# Autodesk Inventor assembly: axis5_6
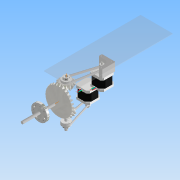
[picture p0: Inventor's stored thumbnail of the model, 180x180]
Saved by Autodesk Inventor 2020 (Build 240168000, 168)
## iProperties
Created: 2020-05-15
Part Number: axis5_6
Document SubType Name: Assembly
Designer: stefa
Author: stefa
## Documents named in this file (12)
- D:\github_gedeeld\BeerMinder\3D-model\axis5_6\axis5_6.iam
- D:\github_gedeeld\BeerMinder\3D-model\pulleys\tandriem32Tnaar16T_lengte240.ipt
- D:\github_gedeeld\BeerMinder\3D-model\pulleys\GT2 Timing Pulley 36T - 8mm as.ipt
- D:\github_gedeeld\BeerMinder\3D-model\stepper motors\42BYG Stepper Motor.ipt
- D:\github_gedeeld\BeerMinder\3D-model\pulleys\GT2 Pulley 16T - 5mm as.ipt
- D:\github_gedeeld\BeerMinder\3D-model\axis5_6\as_d8_l100.ipt
- D:\github_gedeeld\BeerMinder\3D-model\axis5_6\axis5_6\Design Accelerator\Bevel Gears1.iam
- D:\github_gedeeld\BeerMinder\3D-model\axis5_6\endeffector mount part.ipt
- D:\github_gedeeld\BeerMinder\3D-model\axis5_6\bovenarm - links.ipt
- D:\github_gedeeld\BeerMinder\3D-model\axis5_6\as naar endeffector.ipt
- D:\github_gedeeld\BeerMinder\3D-model\axis5_6\stepper spacer.ipt
- D:\github_gedeeld\BeerMinder\3D-model\axis5_6\axis5_6\Design Accelerator\Bevel Gear11.ipt
## Components (15 placed, 11 different names)
1. tandriem32Tnaar16T_lengte240:1 — Mate:5, Mate:6, Mate:21, Mate:22
2. GT2 Pulley 16T - 5mm as:1 — Mate:5, Mate:6, Mate:15, Mate:16
3. as_d8_l100:1 — Mate:20, Mate:23, Mate:26
4. tandriem32Tnaar16T_lengte240:2 — Mate:24, Mate:25
5. GT2 Pulley 16T - 5mm as:2 — Mate:17, Mate:18
6. Bevel Gears:1 [sub-assembly] — Mate:26, Mate:28, Mate:38, Mate:39
7. 42BYG Stepper Motor:2 — Mate:15, Mate:16, Flush:1, Mate:19, Mate:32, Angle:2, Mate:33, Mate:35, Mate:36, Mate:37
8. 42BYG Stepper Motor:3 — Mate:17, Mate:18, Flush:1, Mate:19, Angle:1
9. GT2 Timing Pulley 36T - 8mm as:3 — Mate:23, Mate:24, Mate:25
10. GT2 Timing Pulley 36T - 8mm as:4 — Mate:20, Mate:21, Mate:22
11. endeffector mount part:1 — Mate:27
12. bovenarm - links:1 — Mate:32, Angle:2, Mate:33, Angle:3, Mate:34
13. as naar endeffector:1 — Mate:27, Mate:28, Mate:29, Mate:30, Mate:31, Angle:1
14. stepper spacer:1 — Mate:34, Mate:35, Mate:36, Mate:37
15. Bevel Gear1:1 — Mate:38, Mate:39
## Relationships (33: Mate 29, Angle 3, Flush 1)
- Mate:5: tandriem32Tnaar16T_lengte240:1 ↔ GT2 Pulley 16T - 5mm as:1
- Mate:6 (0.5 mm): tandriem32Tnaar16T_lengte240:1 ↔ GT2 Pulley 16T - 5mm as:1
- [Mate]: tandriem32Tnaar16T_lengte240:2 ↔ GT2 Pulley 16T - 5mm as:2
- [Mate] (0.5 mm): tandriem32Tnaar16T_lengte240:2 ↔ GT2 Pulley 16T - 5mm as:2
- Mate:15: GT2 Pulley 16T - 5mm as:1 ↔ 42BYG Stepper Motor:2
- Mate:16 (2 mm): GT2 Pulley 16T - 5mm as:1 ↔ 42BYG Stepper Motor:2
- Mate:17 (2 mm): GT2 Pulley 16T - 5mm as:2 ↔ 42BYG Stepper Motor:3
- Mate:18: GT2 Pulley 16T - 5mm as:2 ↔ 42BYG Stepper Motor:3
- Flush:1: 42BYG Stepper Motor:2 ↔ 42BYG Stepper Motor:3
- Mate:19 (2 mm): 42BYG Stepper Motor:2 ↔ 42BYG Stepper Motor:3
- Mate:20: as_d8_l100:1 ↔ GT2 Timing Pulley 36T - 8mm as:4
- Mate:21: tandriem32Tnaar16T_lengte240:1 ↔ GT2 Timing Pulley 36T - 8mm as:4
- Mate:22 (0.5 mm): tandriem32Tnaar16T_lengte240:1 ↔ GT2 Timing Pulley 36T - 8mm as:4
- Mate:23: as_d8_l100:1 ↔ GT2 Timing Pulley 36T - 8mm as:3
- Mate:24: tandriem32Tnaar16T_lengte240:2 ↔ GT2 Timing Pulley 36T - 8mm as:3
- Mate:25 (0.5 mm): tandriem32Tnaar16T_lengte240:2 ↔ GT2 Timing Pulley 36T - 8mm as:3
- Mate:26: as_d8_l100:1 ↔ Bevel Gears:1
- Mate:27: endeffector mount part:1 ↔ as naar endeffector:1
- Mate:28: Bevel Gears:1 ↔ as naar endeffector:1
- Mate:29: as naar endeffector:1
- Mate:30: as naar endeffector:1
- Mate:31: as naar endeffector:1
- Angle:1 (0 deg): 42BYG Stepper Motor:3 ↔ as naar endeffector:1
- Mate:32: 42BYG Stepper Motor:2 ↔ bovenarm - links:1
- Angle:2 (0 deg): 42BYG Stepper Motor:2 ↔ bovenarm - links:1
- Mate:33: 42BYG Stepper Motor:2 ↔ bovenarm - links:1
- Angle:3 (0 deg): bovenarm - links:1
- Mate:34: bovenarm - links:1 ↔ stepper spacer:1
- Mate:35: 42BYG Stepper Motor:2 ↔ stepper spacer:1
- Mate:36: 42BYG Stepper Motor:2 ↔ stepper spacer:1
- Mate:37: 42BYG Stepper Motor:2 ↔ stepper spacer:1
- Mate:38: Bevel Gears:1 ↔ Bevel Gear1:1
- Mate:39 (26.661 mm): Bevel Gears:1 ↔ Bevel Gear1:1
## Named parameters: d13_d6 = 0 mm, d14_d7 = 0.5 mm
